# Autodesk Inventor assembly: finalassembly
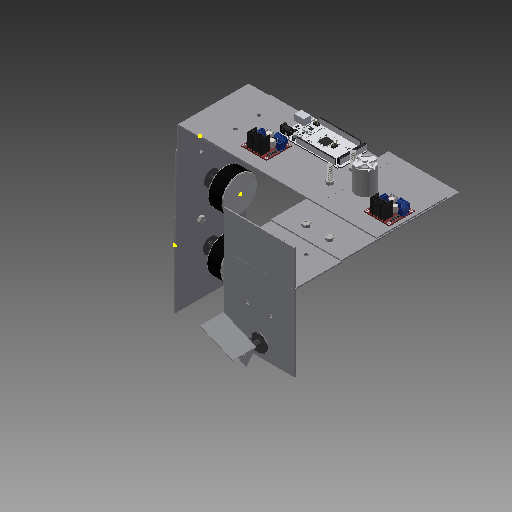
[picture p0: Inventor's stored thumbnail of the model, 512x512]
Saved by Autodesk Inventor 2019 (Build 230136000, 136)
## iProperties
Created: 2020-02-15
Part Number: finalassembly
Document SubType Name: Assembly
Designer: Dell
Author: Dell
## Documents named in this file (5)
- C:\Users\Dell\Documents\finalassembly.iam
- C:\Users\Dell\Documents\Assembly5.iam
- C:\Users\Dell\Documents\anglechangefinal.iam
- C:\Users\Dell\Documents\movementfinal.iam
- C:\Users\Dell\Documents\strikingfinal.iam
## Components (4 placed, 4 different names)
1. Assembly5:1 [sub-assembly] — Rigid:1, Rotational:1, Rotational:7
2. anglechangefinal:1 [sub-assembly] — Rigid:1, Rotational:8
3. movementfinal:1 [sub-assembly] — Rotational:1, Rotational:7
4. strikingfinal:1 [sub-assembly] — Rotational:8
## Relationships (4: RevoluteJoint 3, WeldJoint 1)
- Rigid:1 [WeldJoint]: Assembly5:1 ↔ anglechangefinal:1
- Rotational:1 [RevoluteJoint]: Assembly5:1 ↔ movementfinal:1
- Rotational:7 [RevoluteJoint]: Assembly5:1 ↔ movementfinal:1
- Rotational:8 [RevoluteJoint]: anglechangefinal:1 ↔ strikingfinal:1
